# Autodesk Inventor assembly: PoleHeightMarker
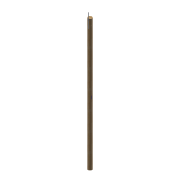
[picture p0: Inventor's stored thumbnail of the model, 180x180]
Saved by Autodesk Inventor 2017 (Build 210142000, 142)
## iProperties
Created: 2017-01-27
Part Number: PoleHeightMarker
Document SubType Name: Assembly
Designer: krosie
Author: krosie
## Documents named in this file (4)
- C:\Users\krosie\Google Drive\HERA\hera-cad\jigs\PoleHeightMarker.iam
- C:\Users\krosie\Google Drive\HERA\hera-cad\support\pole\pole.ipt
- C:\Users\krosie\Google Drive\HERA\hera-cad\feed\bpSupArm.ipt
- C:\Users\krosie\Google Drive\HERA\hera-cad\jigs\PoleHeightMarker.ipt
## Components (3 placed, 3 different names)
1. pole:1 — Flush:1, Tangent:1, Tangent:2, Flush:2
2. bpSupArm:1 — Flush:1, Tangent:1, Mate:1
3. PoleHeightMarker:1 — Mate:1, Tangent:2, Flush:2
## Relationships (5: Flush 2, Tangent 2, Mate 1)
- Flush:1 (-300 mm): pole:1 ↔ bpSupArm:1
- Tangent:1: pole:1 ↔ bpSupArm:1
- Mate:1: bpSupArm:1 ↔ PoleHeightMarker:1
- Tangent:2: pole:1 ↔ PoleHeightMarker:1
- Flush:2 (30 mm): pole:1 ↔ PoleHeightMarker:1
